# Autodesk Inventor assembly: コックピット_1
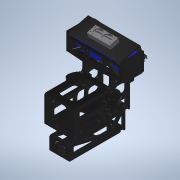
[picture p0: Inventor's stored thumbnail of the model, 180x180]
Saved by Autodesk Inventor 2020 (Build 240168000, 168)
## iProperties
Created: 2016-05-08
Part Number: コックピット_1
Document SubType Name: Assembly
Designer: hiroaki
Mass: 505.272 g
Surface Area: 1895.72 cm^2
Volume: 344.131 cm^3
Density: 1.46825 g/cm^3
Author: hiroaki
## Documents named in this file (25)
- C:\Users\masato\Documents\GitHub\OpenPlatform\mechanism\OpenPlatform_ver3_0\上半身\コックピット\コックピット_2\コックピット_2.iam
- C:\Users\masato\Documents\GitHub\OpenPlatform\mechanism\OpenPlatform_ver3_0\既製品\バッテリー(G7 HI-VOLTAGE 2400MAH 3S 75CMAX LIPO).ipt
- C:\Users\masato\Documents\GitHub\OpenPlatform\mechanism\OpenPlatform_ver3_0\既製品\sw.ipt
- C:\Users\masato\Documents\GitHub\OpenPlatform\mechanism\OpenPlatform_ver3_0\上半身\コックピット\コックピット_2\コックピット_サブフレーム_1_3.ipt
- C:\Users\masato\Documents\GitHub\OpenPlatform\mechanism\OpenPlatform_ver3_0\上半身\コックピット\コックピット_2\コックピット_サブフレーム_1_5.ipt
- C:\Users\masato\Documents\GitHub\OpenPlatform\mechanism\OpenPlatform_ver3_0\上半身\コックピット\コックピット_2\コックピット_サブフレーム_1_6.ipt
- C:\Users\masato\Documents\GitHub\OpenPlatform\mechanism\OpenPlatform_ver3_0\上半身\コックピット\コックピット_2\コックピット_サブフレーム_1_7.ipt
- C:\Users\masato\Documents\GitHub\OpenPlatform\mechanism\OpenPlatform_ver3_0\上半身\コックピット\コックピット_2\コックピット_2_メインフレーム_1.ipt
- C:\Users\masato\Documents\GitHub\OpenPlatform\mechanism\OpenPlatform_ver3_0\上半身\コックピット\コックピット_2\コックピット_2_メインフレーム_1_MIR.ipt
- C:\Users\masato\Documents\GitHub\OpenPlatform\mechanism\OpenPlatform_ver3_0\上半身\コックピット\コックピット_2\コックピット_2_サブフレーム_1.ipt
- C:\Users\masato\Documents\GitHub\OpenPlatform\mechanism\OpenPlatform_ver3_0\上半身\コックピット\コックピット_2\コックピット_2_サブフレーム_2.ipt
- C:\Users\masato\Documents\GitHub\OpenPlatform\mechanism\OpenPlatform_ver3_0\上半身\コックピット\コックピット_2\コックピット_2_サブフレーム_4.ipt
- C:\Users\masato\Documents\GitHub\OpenPlatform\mechanism\OpenPlatform_ver3_0\上半身\コックピット\コックピット_2\コックピット_2_メインフレーム_2.ipt
- C:\Users\masato\Documents\GitHub\OpenPlatform\mechanism\OpenPlatform_ver3_0\上半身\コックピット\コックピット_2\コックピット_2_サブフレーム_5.ipt
- C:\Users\masato\Documents\GitHub\OpenPlatform\mechanism\OpenPlatform_ver3_0\上半身\コックピット\コックピット_2\コックピット_2_サブフレーム_6.ipt
- C:\Users\masato\Documents\GitHub\OpenPlatform\mechanism\OpenPlatform_ver3_0\上半身\コックピット\コックピット_2\コックピット_サブフレーム_1_5_MIR.ipt
- C:\Users\masato\Documents\GitHub\OpenPlatform\mechanism\OpenPlatform_ver3_0\上半身\コックピット\コックピット_2\CIT_OP_J120_Mount.ipt
- C:\Users\masato\Documents\GitHub\OpenPlatform\mechanism\OpenPlatform_ver3_0\上半身\コックピット\コックピット_2\SwitchCov.ipt
- C:\Users\masato\Documents\GitHub\OpenPlatform\mechanism\OpenPlatform_ver3_0\上半身\コックピット\コックピット_2\コックピット_2_メインフレーム_2_MIR.ipt
- C:\Users\masato\Documents\GitHub\OpenPlatform\mechanism\OpenPlatform_ver3_0\上半身\コックピット\コックピット_2\New_Accelite_Controller_Cover_copy_under.ipt
- C:\Users\masato\Documents\GitHub\OpenPlatform\mechanism\OpenPlatform_ver3_0\上半身\コックピット\コックピット_2\New_Accelite_Controller_Cover_copy.ipt
- C:\Users\masato\Documents\GitHub\OpenPlatform\mechanism\OpenPlatform_ver3_0\上半身\コックピット\コックピット_2\Antenna.ipt
- C:\Users\masato\Documents\GitHub\OpenPlatform\mechanism\OpenPlatform_ver3_0\上半身\コックピット\コックピット_2\Antenna_MIR.ipt
- C:\Users\masato\Documents\GitHub\OpenPlatform\mechanism\OpenPlatform_ver3_0\上半身\コックピット\コックピット_2\コックピット_スライドロックカバー.ipt
- C:\Users\masato\Documents\GitHub\OpenPlatform\mechanism\OpenPlatform_ver3_0\上半身\コックピット\コックピット_2\コックピット_スライドロック.ipt
## Components (25 placed, 24 different names)
1. バッテリー(G7 HI-VOLTAGE 2400MAH 3S 75CMAX LIPO):1 — メイト:8, メイト:12, メイト:65
2. sw:1 — フラッシュ:8, フラッシュ:9, メイト:20, メイト:21, メイト:22
3. sw:2 — フラッシュ:8, フラッシュ:9, メイト:23
4. コックピット_サブフレーム_1_3:1 — メイト:12, メイト:14, メイト:15, メイト:17, メイト:19, 挿入:40, 挿入:41, 挿入:42, 挿入:43, 挿入:60, 挿入:61
5. コックピット_サブフレーム_1_6:1 — メイト:14, メイト:15, メイト:18, メイト:65
6. コックピット_サブフレーム_1_5:2 — メイト:17, メイト:18, メイト:19, 挿入:23, 正接:1
7. コックピット_サブフレーム_1_7:1 — 挿入:23, 挿入:68, 挿入:69, 挿入:70, 挿入:71, メイト:72
8. コックピット_2_メインフレーム_1:1 — メイト:20, メイト:21, メイト:22, 挿入:40, 挿入:41, メイト:24, メイト:25, メイト:26, メイト:29, メイト:30, メイト:31, メイト:32, 挿入:48, 挿入:49, 挿入:62, 角度:1, メイト:66, メイト:67, メイト:71
9. コックピット_2_メインフレーム_1_MIR:1 — 挿入:42, 挿入:43, メイト:23, メイト:27, メイト:28, メイト:33, 挿入:50, 挿入:51, メイト:68, メイト:69, メイト:70
10. コックピット_2_サブフレーム_1:1 — メイト:24, メイト:25, メイト:26, メイト:27
11. コックピット_2_サブフレーム_2:1 — メイト:28, メイト:29, メイト:30, メイト:31, メイト:32, メイト:33, 挿入:54, 挿入:55, 挿入:63, 挿入:64, 挿入:67
12. コックピット_2_サブフレーム_4:1 — 挿入:48, 挿入:49, 挿入:50, 挿入:51
13. コックピット_2_メインフレーム_2:1 — 挿入:54, 挿入:55, 挿入:56, 挿入:57, メイト:59, メイト:61
14. コックピット_2_サブフレーム_5:1 — メイト:59, メイト:60, メイト:61
15. コックピット_2_サブフレーム_6:1 — 挿入:56, 挿入:57, 挿入:65, 挿入:66, メイト:60
16. コックピット_サブフレーム_1_5_MIR:1 — 挿入:60, 挿入:61
17. CIT_OP_J120_Mount:1 — 挿入:63, 挿入:64
18. SwitchCov:1 — 挿入:62, 角度:1
19. コックピット_2_メインフレーム_2_MIR:1 — 挿入:65, 挿入:66, 挿入:67
20. New_Accelite_Controller_Cover_copy_under:1 — メイト:62, メイト:63, メイト:64, 挿入:68, 挿入:69
21. New_Accelite_Controller_Cover_copy:1 — メイト:62, メイト:63, メイト:64
22. Antenna:1 — メイト:68, メイト:69, メイト:70
23. Antenna_MIR:1 — メイト:66, メイト:67, メイト:71
24. コックピット_スライドロックカバー:1 — 挿入:70, 挿入:71, 角度:2, 円柱状:1
25. コックピット_スライドロック:1 — メイト:72, 角度:2, 円柱状:1, 正接:1
## Relationships (66: Mate 35, Insert 25, Flush 2, Angle 2, CylindricalJoint 1, Tangent 1)
- メイト:8 [Mate] (-57.5 mm): バッテリー(G7 HI-VOLTAGE 2400MAH 3S 75CMAX LIPO):1
- メイト:12 [Mate] (1 mm): バッテリー(G7 HI-VOLTAGE 2400MAH 3S 75CMAX LIPO):1 ↔ コックピット_サブフレーム_1_3:1
- メイト:14 [Mate] (0.05 mm): コックピット_サブフレーム_1_3:1 ↔ コックピット_サブフレーム_1_6:1
- メイト:15 [Mate]: コックピット_サブフレーム_1_3:1 ↔ コックピット_サブフレーム_1_6:1
- メイト:17 [Mate]: コックピット_サブフレーム_1_3:1 ↔ コックピット_サブフレーム_1_5:2
- メイト:18 [Mate] (0.05 mm): コックピット_サブフレーム_1_6:1 ↔ コックピット_サブフレーム_1_5:2
- メイト:19 [Mate] (0.05 mm): コックピット_サブフレーム_1_3:1 ↔ コックピット_サブフレーム_1_5:2
- 挿入:23 [Insert] (-10 mm): コックピット_サブフレーム_1_5:2 ↔ コックピット_サブフレーム_1_7:1
- フラッシュ:8 [Flush]: sw:1 ↔ sw:2
- フラッシュ:9 [Flush]: sw:1 ↔ sw:2
- メイト:20 [Mate]: sw:1 ↔ コックピット_2_メインフレーム_1:1
- メイト:21 [Mate] (0.55 mm): sw:1 ↔ コックピット_2_メインフレーム_1:1
- メイト:22 [Mate] (0.3 mm): sw:1 ↔ コックピット_2_メインフレーム_1:1
- 挿入:40 [Insert]: コックピット_サブフレーム_1_3:1 ↔ コックピット_2_メインフレーム_1:1
- 挿入:41 [Insert]: コックピット_サブフレーム_1_3:1 ↔ コックピット_2_メインフレーム_1:1
- 挿入:42 [Insert]: コックピット_サブフレーム_1_3:1 ↔ コックピット_2_メインフレーム_1_MIR:1
- 挿入:43 [Insert]: コックピット_サブフレーム_1_3:1 ↔ コックピット_2_メインフレーム_1_MIR:1
- メイト:23 [Mate]: sw:2 ↔ コックピット_2_メインフレーム_1_MIR:1
- メイト:24 [Mate] (0.05 mm): コックピット_2_メインフレーム_1:1 ↔ コックピット_2_サブフレーム_1:1
- メイト:25 [Mate] (0.05 mm): コックピット_2_メインフレーム_1:1 ↔ コックピット_2_サブフレーム_1:1
- メイト:26 [Mate]: コックピット_2_メインフレーム_1:1 ↔ コックピット_2_サブフレーム_1:1
- メイト:27 [Mate]: コックピット_2_メインフレーム_1_MIR:1 ↔ コックピット_2_サブフレーム_1:1
- メイト:28 [Mate]: コックピット_2_メインフレーム_1_MIR:1 ↔ コックピット_2_サブフレーム_2:1
- メイト:29 [Mate]: コックピット_2_メインフレーム_1:1 ↔ コックピット_2_サブフレーム_2:1
- メイト:30 [Mate] (0.05 mm): コックピット_2_メインフレーム_1:1 ↔ コックピット_2_サブフレーム_2:1
- メイト:31 [Mate] (0.05 mm): コックピット_2_メインフレーム_1:1 ↔ コックピット_2_サブフレーム_2:1
- メイト:32 [Mate] (0.05 mm): コックピット_2_メインフレーム_1:1 ↔ コックピット_2_サブフレーム_2:1
- メイト:33 [Mate] (0.05 mm): コックピット_2_メインフレーム_1_MIR:1 ↔ コックピット_2_サブフレーム_2:1
- 挿入:48 [Insert]: コックピット_2_メインフレーム_1:1 ↔ コックピット_2_サブフレーム_4:1
- 挿入:49 [Insert]: コックピット_2_メインフレーム_1:1 ↔ コックピット_2_サブフレーム_4:1
- 挿入:50 [Insert]: コックピット_2_メインフレーム_1_MIR:1 ↔ コックピット_2_サブフレーム_4:1
- 挿入:51 [Insert]: コックピット_2_メインフレーム_1_MIR:1 ↔ コックピット_2_サブフレーム_4:1
- 挿入:54 [Insert]: コックピット_2_サブフレーム_2:1 ↔ コックピット_2_メインフレーム_2:1
- 挿入:55 [Insert]: コックピット_2_サブフレーム_2:1 ↔ コックピット_2_メインフレーム_2:1
- 挿入:56 [Insert]: コックピット_2_メインフレーム_2:1 ↔ コックピット_2_サブフレーム_6:1
- 挿入:57 [Insert]: コックピット_2_メインフレーム_2:1 ↔ コックピット_2_サブフレーム_6:1
- 挿入:60 [Insert]: コックピット_サブフレーム_1_3:1 ↔ コックピット_サブフレーム_1_5_MIR:1
- 挿入:61 [Insert]: コックピット_サブフレーム_1_3:1 ↔ コックピット_サブフレーム_1_5_MIR:1
- 挿入:62 [Insert]: コックピット_2_メインフレーム_1:1 ↔ SwitchCov:1
- 挿入:63 [Insert]: コックピット_2_サブフレーム_2:1 ↔ CIT_OP_J120_Mount:1
- 角度:1 [Angle] (180 deg): コックピット_2_メインフレーム_1:1 ↔ SwitchCov:1
- 挿入:64 [Insert]: コックピット_2_サブフレーム_2:1 ↔ CIT_OP_J120_Mount:1
- 挿入:65 [Insert]: コックピット_2_サブフレーム_6:1 ↔ コックピット_2_メインフレーム_2_MIR:1
- 挿入:66 [Insert]: コックピット_2_サブフレーム_6:1 ↔ コックピット_2_メインフレーム_2_MIR:1
- 挿入:67 [Insert]: コックピット_2_サブフレーム_2:1 ↔ コックピット_2_メインフレーム_2_MIR:1
- メイト:59 [Mate]: コックピット_2_メインフレーム_2:1 ↔ コックピット_2_サブフレーム_5:1
- メイト:60 [Mate]: コックピット_2_サブフレーム_5:1 ↔ コックピット_2_サブフレーム_6:1
- メイト:61 [Mate] (0.05 mm): コックピット_2_メインフレーム_2:1 ↔ コックピット_2_サブフレーム_5:1
- メイト:62 [Mate]: New_Accelite_Controller_Cover_copy_under:1 ↔ New_Accelite_Controller_Cover_copy:1
- メイト:63 [Mate]: New_Accelite_Controller_Cover_copy_under:1 ↔ New_Accelite_Controller_Cover_copy:1
- メイト:64 [Mate]: New_Accelite_Controller_Cover_copy_under:1 ↔ New_Accelite_Controller_Cover_copy:1
- 挿入:68 [Insert]: コックピット_サブフレーム_1_7:1 ↔ New_Accelite_Controller_Cover_copy_under:1
- 挿入:69 [Insert]: コックピット_サブフレーム_1_7:1 ↔ New_Accelite_Controller_Cover_copy_under:1
- メイト:65 [Mate] (6 mm): バッテリー(G7 HI-VOLTAGE 2400MAH 3S 75CMAX LIPO):1 ↔ コックピット_サブフレーム_1_6:1
- メイト:66 [Mate]: コックピット_2_メインフレーム_1:1 ↔ Antenna_MIR:1
- メイト:67 [Mate]: コックピット_2_メインフレーム_1:1 ↔ Antenna_MIR:1
- メイト:68 [Mate]: コックピット_2_メインフレーム_1_MIR:1 ↔ Antenna:1
- メイト:69 [Mate]: コックピット_2_メインフレーム_1_MIR:1 ↔ Antenna:1
- メイト:70 [Mate] (4 mm): コックピット_2_メインフレーム_1_MIR:1 ↔ Antenna:1
- メイト:71 [Mate] (4 mm): コックピット_2_メインフレーム_1:1 ↔ Antenna_MIR:1
- 挿入:70 [Insert]: コックピット_サブフレーム_1_7:1 ↔ コックピット_スライドロックカバー:1
- 挿入:71 [Insert]: コックピット_サブフレーム_1_7:1 ↔ コックピット_スライドロックカバー:1
- メイト:72 [Mate]: コックピット_サブフレーム_1_7:1 ↔ コックピット_スライドロック:1
- 角度:2 [Angle] (0 deg): コックピット_スライドロックカバー:1 ↔ コックピット_スライドロック:1
- 円柱状:1 [CylindricalJoint]: コックピット_スライドロックカバー:1 ↔ コックピット_スライドロック:1
- 正接:1 [Tangent]: コックピット_サブフレーム_1_5:2 ↔ コックピット_スライドロック:1
